# Autodesk Inventor assembly: 6 HiGrip with hub and double pulley
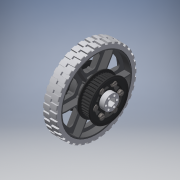
[picture p0: Inventor's stored thumbnail of the model, 180x180]
Saved by Autodesk Inventor 2017.1 (Build 211199000, 199)
## iProperties
Created: 2015-12-05
Part Number: 6 HiGrip with hub and double pulley
Document SubType Name: Assembly
Designer: PhillipD
Author: PhillipD
Revision Number: ANY
## Documents named in this file (6)
- D:\FIRST\FIRST KOP 2017\FIRST Drive Base\Parts\6 HiGrip with hub and double pulley.iam
- D:\FIRST\FIRST KOP 2017\FIRST Drive Base\Parts\6 HiGrip Asm Rev III.iam
- D:\FIRST\FIRST KOP 2017\FIRST Drive Base\Parts\42 tooth HTD Pulley half 2014.ipt
- D:\FIRST\FIRST KOP 2017\FIRST Drive Base\Parts\10-24 Hex Washer Rolling x 1.25_93882A213.ipt
- D:\FIRST\FIRST KOP 2017\FIRST Drive Base\Parts\500EX Hex Hub.ipt
- D:\FIRST\FIRST KOP 2017\FIRST Drive Base\Parts\am-1305 500 Hex Spacer.ipt
## Components (19 placed, 19 different names)
1. 6 HiGrip Asm Rev II_46 [sub-assembly]
2. 42 tooth HTD Pulley half 2014_47
3. 42 tooth HTD Pulley half 2014_48 — Insert:1
4. 10-24 Hex Washer Rolling x 1.25_93882A213_49
5. 10-24 Hex Washer Rolling x 1.25_93882A213_50
6. 10-24 Hex Washer Rolling x 1.25_93882A213_51
7. 10-24 Hex Washer Rolling x 1.25_93882A213_52
8. 10-24 Hex Washer Rolling x 1.25_93882A213_53
9. 10-24 Hex Washer Rolling x 1.25_93882A213_54
10. 42 tooth HTD Pulley half 2014_55
11. 42 tooth HTD Pulley half 2014_56
12. 500EX Hex Hub_57
13. 10-24 Hex Washer Rolling x 1.25_93882A213_58
14. 10-24 Hex Washer Rolling x 1.25_93882A213_59
15. 10-24 Hex Washer Rolling x 1.25_93882A213_60
16. 10-24 Hex Washer Rolling x 1.25_93882A213_61
17. 10-24 Hex Washer Rolling x 1.25_93882A213_62
18. 10-24 Hex Washer Rolling x 1.25_93882A213_63
19. am-1305 500 Hex Spacer_64 — Insert:1
## Relationships (1: Insert 1)
- Insert:1: 42 tooth HTD Pulley half 2014_48 ↔ am-1305 500 Hex Spacer_64
